# Autodesk Inventor assembly: Ensamblaje1
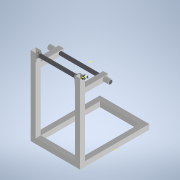
[picture p0: Inventor's stored thumbnail of the model, 180x180]
Saved by Autodesk Inventor 2021 (Build 250183000, 183)
## iProperties
Created: 2022-02-18
Part Number: Ensamblaje1
Document SubType Name: Assembly
Designer: arthu
Author: arthu
## Documents named in this file (6)
- C:\Users\arthu\OneDrive\Escritorio\Bloquera\Ensamblaje1.iam
- C:\Users\arthu\OneDrive\Escritorio\Bloquera\Principal.ipt
- C:\Users\arthu\OneDrive\Escritorio\Bloquera\tubo_2pul_1.ipt
- C:\Users\arthu\OneDrive\Escritorio\Bloquera\acople_2pulg.ipt
- C:\Users\arthu\OneDrive\Escritorio\Bloquera\chumacera.ipt
- C:\Users\arthu\OneDrive\Escritorio\Bloquera\tubo_2pul_2.ipt
## Components (7 placed, 5 different names)
1. Principal:1 — Insertar:1, De rotación:1, De rotación:2
2. tubo_2pul_1:1 — Insertar:1, Insertar:2, Insertar:3
3. acople_2pulg:1 — Insertar:2
4. acople_2pulg:2 — Insertar:3
5. chumacera:1 — De rotación:1
6. chumacera:2 — De rotación:2, Insertar:4
7. tubo_2pul_2:1 — Insertar:4
## Relationships (6: Insert 4, RevoluteJoint 2)
- Insertar:1 (-850 mm): Principal:1 ↔ tubo_2pul_1:1
- Insertar:2: tubo_2pul_1:1 ↔ acople_2pulg:1
- Insertar:3: tubo_2pul_1:1 ↔ acople_2pulg:2
- De rotación:1 [RevoluteJoint]: Principal:1 ↔ chumacera:1
- De rotación:2 [RevoluteJoint]: Principal:1 ↔ chumacera:2
- Insertar:4 (-26 mm): chumacera:2 ↔ tubo_2pul_2:1
